# Autodesk Inventor assembly: PayloadGermination
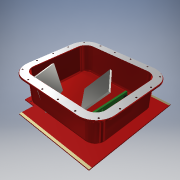
[picture p0: Inventor's stored thumbnail of the model, 180x180]
Saved by Autodesk Inventor 2018 (Build 220112000, 112)
## iProperties
Created: 2018-07-04
Part Number: PayloadGermination
Document SubType Name: Assembly
Designer: Bradley
Mass: 94.7116 g
Surface Area: 468.462 cm^2
Volume: 39.9332 cm^3
Density: 2.37175 g/cm^3
Author: Bradley
## Documents named in this file (5)
- D:\Users\Bradley\Documents\CougsInSpace\CougSat1-Hardware\CougSat1-Payload\CADModel\Native\PayloadGermination.iam
- D:\Users\Bradley\Documents\CougsInSpace\CougSat1-Hardware\CougSat1-Payload\CADModel\Native\PayloadGermination_PCB.ipt
- D:\Users\Bradley\Documents\CougsInSpace\CougSat1-Hardware\CougSat1-Payload\CADModel\Native\PayloadGermination_Chamber.ipt
- D:\Users\Bradley\Documents\CougsInSpace\Resources\ComponentModels\Electronics\Module_ArducamMini.ipt
- D:\Users\Bradley\Documents\CougsInSpace\CougSat1-Hardware\CougSat1-Payload\CADModel\Native\PayloadGermination_Mirror.ipt
## Components (5 placed, 4 different names)
1. PayloadGermination_PCB:1
2. PayloadGermination_Chamber:1 — Flush:1, Flush:2, Flush:3, Mate:1, Mate:2
3. Module_ArducamMini:1 — Mate:1, Mate:2
4. PayloadGermination_Mirror:1
5. PayloadGermination_Mirror:2
## Relationships (5: Flush 3, Mate 2)
- Flush:1: PayloadGermination_Chamber:1
- Flush:2 (-31.5 mm): PayloadGermination_Chamber:1
- Flush:3 (44.4 mm): PayloadGermination_Chamber:1
- Mate:1: PayloadGermination_Chamber:1 ↔ Module_ArducamMini:1
- Mate:2 (5 mm): PayloadGermination_Chamber:1 ↔ Module_ArducamMini:1
